# Autodesk Inventor assembly: wheel_hub
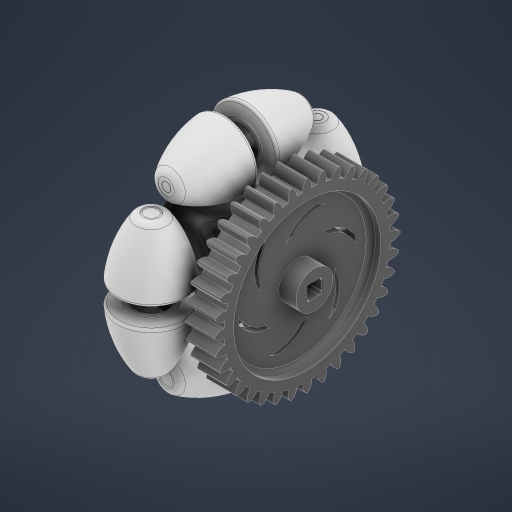
[picture p0: Inventor's stored thumbnail of the model, 512x512]
Saved by Autodesk Inventor 2024 (Build 280153000, 153)
## iProperties
Created: 2024-01-13
Part Number: wheel_hub
Document SubType Name: Assembly
Designer: avere
Author: avere
## Documents named in this file (3)
- C:\Users\avere\Documents\rbp_cad\zoomba_v0.3\wheel_hub.iam
- C:\Users\avere\Documents\rbp_cad\VEX-CAD-Inventor-1.41\Motion\Wheels\Omni Wheel\2” Omni-Directional Wheel (276-9044)\2” Omni-Directional Wheel (276-9044).ipt
- C:\Users\avere\Documents\rbp_cad\VEX-CAD-Inventor-1.41\Motion\Gears\LS 36T Gear.ipt
## Components (2 placed, 2 different names)
1. 2” Omni-Directional Wheel (276-9044):1 — Insert:1
2. LS 36T Gear:1 — Insert:1
## Relationships (1: Insert 1)
- Insert:1: 2” Omni-Directional Wheel (276-9044):1 ↔ LS 36T Gear:1
